# Autodesk Inventor assembly: Claw Assembly
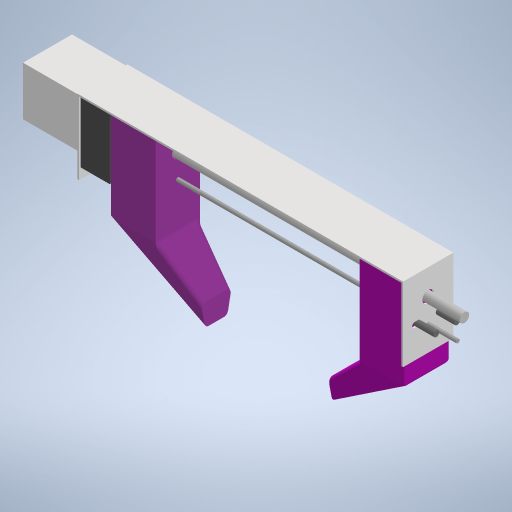
[picture p0: Inventor's stored thumbnail of the model, 512x512]
Saved by Autodesk Inventor 2024 (Build 280153000, 153)
## iProperties
Created: 2025-01-21
Part Number: Claw Assembly
Document SubType Name: Assembly
Designer: Sven
Author: Sven
## Documents named in this file (10)
- C:\Users\Sven\Documents\Inventor\BRC Robotic CLaw\Claw Assembly.iam
- C:\Users\Sven\Documents\Inventor\BRC Robotic CLaw\Bracket.ipt
- C:\Users\Sven\Documents\Inventor\BRC Robotic CLaw\Moving Gripper.ipt
- C:\Users\Sven\Documents\Inventor\BRC Robotic CLaw\Stationary Gripper.ipt
- C:\Users\Sven\Documents\Inventor\BRC Robotic CLaw\Lead Screw.ipt
- C:\Users\Sven\Documents\Inventor\BRC Robotic CLaw\#10 2in.ipt
- C:\Users\Sven\Documents\Inventor\BRC Robotic CLaw\Support Bar.ipt
- C:\Users\Sven\Documents\Inventor\BRC Robotic CLaw\Motor Brace.ipt
- C:\Users\Sven\Documents\Inventor\BRC Robotic CLaw\Couple.ipt
- C:\Users\Sven\Documents\Inventor\BRC Robotic CLaw\NEMA 17 Completely Correct.ipt
## Components (10 placed, 9 different names)
1. Bracket:1 — Mate:3, Mate:4, Mate:5, Mate:12, Mate:15, Flush:2, Mate:16, Mate:17, Mate:18, Mate:22, Mate:23, Mate:26
2. Moving Gripper:1 — Mate:5, Mate:6, Mate:14, Mate:19
3. Stationary Gripper:1 — Mate:4, Mate:7, Mate:8, Mate:9, Mate:10, Mate:11, Mate:12, Mate:14
4. Lead Screw:1 — Mate:3, Mate:6, Mate:7, Mate:20, Mate:21, Mate:25
5. #10 2in:1 — Mate:8, Mate:9
6. #10 2in:2 — Mate:10, Mate:11
7. Support Bar:1 — Mate:15, Flush:2
8. Motor Brace:1 — Mate:16, Mate:17, Mate:18, Mate:19
9. Couple:1 — Mate:20, Mate:21, Mate:24
10. NEMA 17 Completely Correct:1 — Mate:22, Mate:23, Mate:24, Mate:25, Mate:26
## Relationships (24: Mate 23, Flush 1)
- Mate:3: Bracket:1 ↔ Lead Screw:1
- Mate:4: Bracket:1 ↔ Stationary Gripper:1
- Mate:5: Bracket:1 ↔ Moving Gripper:1
- Mate:6: Moving Gripper:1 ↔ Lead Screw:1
- Mate:7: Stationary Gripper:1 ↔ Lead Screw:1
- Mate:8: Stationary Gripper:1 ↔ #10 2in:1
- Mate:9: Stationary Gripper:1 ↔ #10 2in:1
- Mate:10: Stationary Gripper:1 ↔ #10 2in:2
- Mate:11: Stationary Gripper:1 ↔ #10 2in:2
- Mate:12: Bracket:1 ↔ Stationary Gripper:1
- Mate:14: Moving Gripper:1 ↔ Stationary Gripper:1
- Mate:15: Bracket:1 ↔ Support Bar:1
- Flush:2: Bracket:1 ↔ Support Bar:1
- Mate:16: Bracket:1 ↔ Motor Brace:1
- Mate:17: Bracket:1 ↔ Motor Brace:1
- Mate:18: Bracket:1 ↔ Motor Brace:1
- Mate:19: Moving Gripper:1 ↔ Motor Brace:1
- Mate:20: Lead Screw:1 ↔ Couple:1
- Mate:21: Lead Screw:1 ↔ Couple:1
- Mate:22: Bracket:1 ↔ NEMA 17 Completely Correct:1
- Mate:23: Bracket:1 ↔ NEMA 17 Completely Correct:1
- Mate:24: Couple:1 ↔ NEMA 17 Completely Correct:1
- Mate:25: Lead Screw:1 ↔ NEMA 17 Completely Correct:1
- Mate:26: Bracket:1 ↔ NEMA 17 Completely Correct:1
